# Autodesk Inventor assembly: Сборка глаза вороны
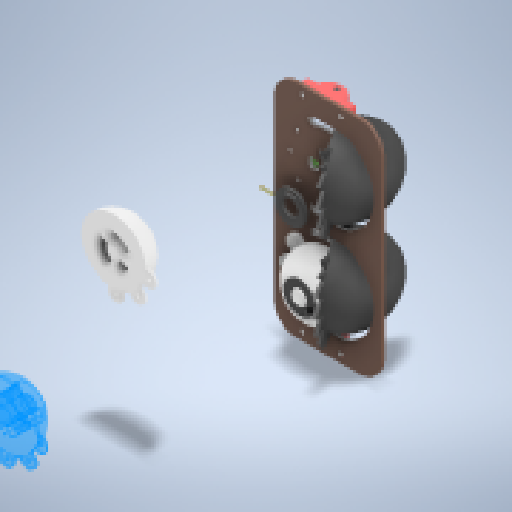
[picture p0: Inventor's stored thumbnail of the model, 512x512]
Saved by Autodesk Inventor 2023.2 (Build 272271030, 271C)
## iProperties
Company: UNSPECIFIED
Created: 1900-01-01
Part Number: Сборка глаза вороны
Description: STEP AP214
Document SubType Name: Assembly
Designer: I9232
Sending System: C3D Toolkit
Preprocessor: C3D Converter
Title: Ñáîðêà ãëàçà âîðîíû
Author: UNSPECIFIED
Revision Number: ANYUNSPECIFIED
## Documents named in this file (14)
- D:\!project\fox_n_crow_construction\crow\face\Сборка глаза вороны.iam
- D:\!project\fox_n_crow_construction\crow\face\Платформа Глаз.ipt
- D:\!project\fox_n_crow_construction\crow\face\Светодиод.ipt
- D:\!project\fox_n_crow_construction\crow\face\Веко правое.ipt
- D:\!project\fox_n_crow_construction\crow\face\MicroServo-SG90.ipt
- D:\!project\fox_n_crow_construction\crow\face\Качалка сервы.ipt
- D:\!project\fox_n_crow_construction\crow\face\Крепление для оси.ipt
- D:\!project\fox_n_crow_construction\crow\face\Крепление для оси_1.ipt
- D:\!project\fox_n_crow_construction\crow\face\M3x4.6x5.ipt
- D:\!project\fox_n_crow_construction\crow\face\Кронштей правый.ipt
- D:\!project\fox_n_crow_construction\crow\face\Кронштей левый.ipt
- D:\!project\fox_n_crow_construction\crow\face\Веко левое.ipt
- D:\!project\fox_n_crow_construction\crow\face\Глаз левый.ipt
- D:\!project\fox_n_crow_construction\crow\face\Глаз правый.ipt
## Components (21 placed, 10 different names)
1. Платформа глаз — Совмещение:2, Совмещение:4, Совмещение:5, Совмещение:11, Совмещение:12, Совмещение:13
2. ANY:2 — Совмещение:9, Совмещение:10
3. ANY:3 — Совмещение:14, Совмещение:15
4. ANY:4
5. ANY:5
6. ANY:6
7. ANY:7
8. Качалка правая
9. Крепление для оси левое
10. Крепление оси правое
11. ANY:11
12. ANY:12
13. ANY:13
14. ANY:14
15. ANY:15
16. ANY:16
17. Кронштеин правый
18. Кронштеин левый
19. Веко левое
20. Глаз левый:1 — Совмещение:2, Совмещение:4, Совмещение:5, Совмещение:9, Совмещение:10
21. Глаз правый:1 — Совмещение:11, Совмещение:12, Совмещение:13, Совмещение:14, Совмещение:15
## Relationships (10: Mate 10)
- Совмещение:2 [Mate]: Платформа глаз ↔ Глаз левый:1
- Совмещение:4 [Mate]: Платформа глаз ↔ Глаз левый:1
- Совмещение:5 [Mate]: Платформа глаз ↔ Глаз левый:1
- Совмещение:9 [Mate]: ANY:2 ↔ Глаз левый:1
- Совмещение:10 [Mate]: ANY:2 ↔ Глаз левый:1
- Совмещение:11 [Mate]: Платформа глаз ↔ Глаз правый:1
- Совмещение:12 [Mate]: Платформа глаз ↔ Глаз правый:1
- Совмещение:13 [Mate]: Платформа глаз ↔ Глаз правый:1
- Совмещение:14 [Mate]: ANY:3 ↔ Глаз правый:1
- Совмещение:15 [Mate]: ANY:3 ↔ Глаз правый:1
